# Autodesk Inventor assembly: gearbox
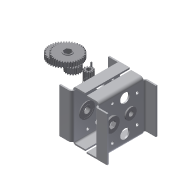
[picture p0: Inventor's stored thumbnail of the model, 180x180]
Saved by Autodesk Inventor 2013 SP1 (Build 170176100, 176)
## iProperties
Created: 2013-12-02
Part Number: gearbox
Document SubType Name: Assembly
Designer: robotics
Author: robotics
## Documents named in this file (9)
- C:\Users\robotics\Documents\GitHub\2014-Preseason-Single-Speed-Gearbox\manufacture\assemblies\gearbox.iam
- C:\Users\robotics\Documents\GitHub\2014-Preseason-Single-Speed-Gearbox\buy\VexPro\Gears\217-2701-STEP\Imported Components\217-2701.20121204\217-2701.20121204.ipt
- C:\Users\robotics\Documents\GitHub\2014-Preseason-Single-Speed-Gearbox\buy\VexPro\Gears\217-2707-STEP\Imported Components\217-2707.20121204\217-2707.20121204.ipt
- C:\Users\robotics\Documents\GitHub\2014-Preseason-Single-Speed-Gearbox\buy\VexPro\Gears\217-2708-STEP\Imported Components\217-2708.20121204\217-2708.20121204.ipt
- C:\Users\robotics\Documents\GitHub\2014-Preseason-Single-Speed-Gearbox\buy\VexPro\Gears\217-2614-Rev02-STEP\Imported Components\217-2614-002\217-2614-002.ipt
- C:\Users\robotics\Documents\GitHub\2014-Preseason-Single-Speed-Gearbox\buy\VexPro\Gears\217-2614-Rev02-STEP\Imported Components\217-2614-001\217-2614-001.ipt
- C:\Users\robotics\Documents\GitHub\2014-Preseason-Single-Speed-Gearbox\buy\VexPro\Gears\217-2614-Rev02-STEP\Imported Components\217-2761-001 rev1\217-2761-001 rev1.ipt
- C:\Users\robotics\Documents\GitHub\2014-Preseason-Single-Speed-Gearbox\manufacture\assemblies\MotorPlate.iam
- C:\Users\robotics\Documents\GitHub\2014-Preseason-Single-Speed-Gearbox\manufacture\assemblies\NonMotorPlate.iam
## Components (8 placed, 8 different names)
1. 217-2701.20121204:1
2. 217-2707.20121204:1
3. 217-2708.20121204:1
4. 217-2614-002:1
5. 217-2614-001:1
6. 217-2761-001 rev1:1
7. MotorPlate:1 [sub-assembly]
8. NonMotorPlate:1 [sub-assembly]
## Relationships (2: Mate 1, Flush 1)
- [Mate]: MotorPlate:1 ↔ NonMotorPlate:1
- [Flush]: MotorPlate:1 ↔ NonMotorPlate:1
